# Autodesk Inventor assembly: BodyNeck_assembly001
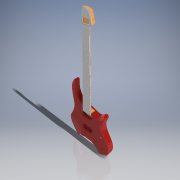
[picture p0: Inventor's stored thumbnail of the model, 180x180]
Saved by Autodesk Inventor 2017 (Build 210142000, 142)
## iProperties
Created: 2016-07-28
Part Number: BodyNeck_assembly001
Document SubType Name: Assembly
Designer: Andy
Author: Andy
## Documents named in this file (3)
- C:\Users\Andy\Desktop\CAD\Guitar\Compass\BodyNeck_assembly001.iam
- C:\Users\Andy\Desktop\CAD\Guitar\Compass\Neck_assembly001.iam
- C:\Users\Andy\Desktop\CAD\Guitar\Compass\rev2.1.ipt
## Components (2 placed, 2 different names)
1. rev2.1:1 — Mate:1, Mate:2, Mate:3
2. Neck_assembly001:1 [sub-assembly] — Mate:1, Mate:2, Mate:3
## Relationships (3: Mate 3)
- Mate:1: rev2.1:1 ↔ Neck_assembly001:1
- Mate:2: rev2.1:1 ↔ Neck_assembly001:1
- Mate:3: rev2.1:1 ↔ Neck_assembly001:1
